# Autodesk Inventor assembly: Assembly
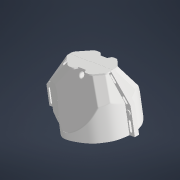
[picture p0: Inventor's stored thumbnail of the model, 180x180]
Saved by Autodesk Inventor 2021 (Build 250183000, 183)
## iProperties
Created: 2020-06-04
Part Number: Assembly
Document SubType Name: Assembly
Designer: Shadow
Author: Shadow
## Documents named in this file (7)
- C:\Users\Shadow\OneDrive - UC San Diego\Projects\PPE\Masks\Valve\Mold_10\Assembly.iam
- C:\Users\Shadow\OneDrive - UC San Diego\Projects\PPE\Masks\Valve\Mask.ipt
- C:\Users\Shadow\OneDrive - UC San Diego\Projects\PPE\Masks\Valve\Mold_10\Core.ipt
- C:\Users\Shadow\OneDrive - UC San Diego\Projects\PPE\Masks\Valve\Mold_10\Left.ipt
- C:\Users\Shadow\OneDrive - UC San Diego\Projects\PPE\Masks\Valve\Mold_10\Press.ipt
- C:\Users\Shadow\OneDrive - UC San Diego\Projects\PPE\Masks\Valve\Mold_10\CorePin.ipt
- C:\Users\Shadow\OneDrive - UC San Diego\Projects\PPE\Masks\Valve\Mold_10\Right.ipt
## Components (8 placed, 6 different names)
1. Mask:1 — Mate:1, Mate:2
2. Core:1 — Flush:1, Flush:2, Flush:4, Mate:3, Mate:4, Flush:5, Flush:6, Cylindrical:1, Cylindrical:2
3. Left:1 — Flush:3, Flush:4
4. Press:1 — Flush:5, Mate:6, Mate:7, Mate:8, Flush:7
5. CorePin:1 — Flush:6, Mate:7
6. CorePin:2 — Cylindrical:2, Mate:6, Mate:8
7. CorePin:3 — Cylindrical:1
8. Right:1 — Flush:7
## Relationships (17: Mate 8, Flush 7, CylindricalJoint 2)
- Flush:1: Core:1
- Flush:2 (40 mm): Core:1
- Flush:3: Left:1
- Flush:4: Core:1 ↔ Left:1
- Mate:1: Mask:1
- Mate:2: Mask:1
- Mate:3: Core:1
- Mate:4: Core:1
- Mate:5
- Flush:5: Core:1 ↔ Press:1
- Flush:6: Core:1 ↔ CorePin:1
- Cylindrical:1: Core:1 ↔ CorePin:3
- Cylindrical:2: Core:1 ↔ CorePin:2
- Mate:6: Press:1 ↔ CorePin:2
- Mate:7: Press:1 ↔ CorePin:1
- Mate:8: Press:1 ↔ CorePin:2
- Flush:7: Press:1 ↔ Right:1
